# Autodesk Inventor assembly: Plant_Home_Alone
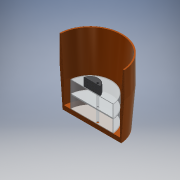
[picture p0: Inventor's stored thumbnail of the model, 180x180]
Saved by Autodesk Inventor 2017 (Build 210142000, 142)
## iProperties
Part Number: Plant_Home_Alone
Material: Generisch
Document SubType Name: Assembly
Designer: OleSi
Author: OleSi
## Documents named in this file (4)
- C:\Users\OleSi\Documents\GitHub\3D_modeling\BWL\Plant_Home_Alone.iam
- C:\Users\OleSi\Documents\GitHub\3D_modeling\BWL\Hub.ipt
- C:\Users\OleSi\Documents\GitHub\3D_modeling\BWL\Tank.ipt
- C:\Users\OleSi\Documents\GitHub\3D_modeling\BWL\Blumentopf.ipt
## Components (4 placed, 3 different names)
1. Hub:1 — Zylindrisch:1, Drehbar:1
2. Tank:1 — Zylindrisch:1, Drehbar:1, Einfügen:1, Passend:1, Passend:2
3. Tank:2 — Einfügen:1, Passend:1, Passend:3
4. Blumentopf:1 — Passend:2, Passend:3
## Relationships (6: Mate 3, CylindricalJoint 1, RevoluteJoint 1, Insert 1)
- Zylindrisch:1 [CylindricalJoint]: Hub:1 ↔ Tank:1
- Drehbar:1 [RevoluteJoint]: Hub:1 ↔ Tank:1
- Einfügen:1 [Insert]: Tank:1 ↔ Tank:2
- Passend:1 [Mate]: Tank:1 ↔ Tank:2
- Passend:2 [Mate]: Tank:1 ↔ Blumentopf:1
- Passend:3 [Mate]: Tank:2 ↔ Blumentopf:1
